# Autodesk Inventor assembly: SlipRingAssy
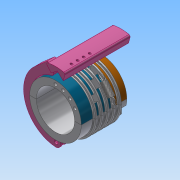
[picture p0: Inventor's stored thumbnail of the model, 180x180]
Saved by Autodesk Inventor 2017.3 (Build 213256000, 256)
## iProperties
Created: 2019-06-19
Part Number: SlipRingAssy
Document SubType Name: Assembly
Designer: Derek Wider
Author: Derek Wider
## Documents named in this file (6)
- G:\Projects\Submarine\Submarine-project\CAD\SlipRing\SlipRingAssy.iam
- G:\Projects\Submarine\Submarine-project\CAD\SlipRing\Core.ipt
- G:\Projects\Submarine\Submarine-project\CAD\SlipRing\CoreOpposite.ipt
- G:\Projects\Submarine\Submarine-project\CAD\SlipRing\ContactMount.ipt
- G:\Projects\Submarine\Submarine-project\CAD\SlipRing\BearingHolder1.ipt
- G:\Projects\Submarine\Submarine-project\CAD\SlipRing\Spring_Extension.ipt
## Components (5 placed, 5 different names)
1. Core:1 — Mate:1, Mate:2, Flush:1, Mate:3, Flush:2
2. CoreOpposite:1 — Mate:1, Mate:2, Flush:1, Mate:4
3. ContactMount:1 — Mate:3, Flush:2, Flush:3, Mate:5
4. BearingHolder1:1 — Mate:4, Flush:3, Mate:5
5. Spring_Extension:1
## Relationships (8: Mate 5, Flush 3)
- Mate:1: Core:1 ↔ CoreOpposite:1
- Mate:2: Core:1 ↔ CoreOpposite:1
- Flush:1: Core:1 ↔ CoreOpposite:1
- Mate:3: Core:1 ↔ ContactMount:1
- Flush:2: Core:1 ↔ ContactMount:1
- Mate:4: CoreOpposite:1 ↔ BearingHolder1:1
- Flush:3 (1.905 mm): ContactMount:1 ↔ BearingHolder1:1
- Mate:5: ContactMount:1 ↔ BearingHolder1:1
